# Autodesk Inventor assembly: ASY PNS-Filter column D1000
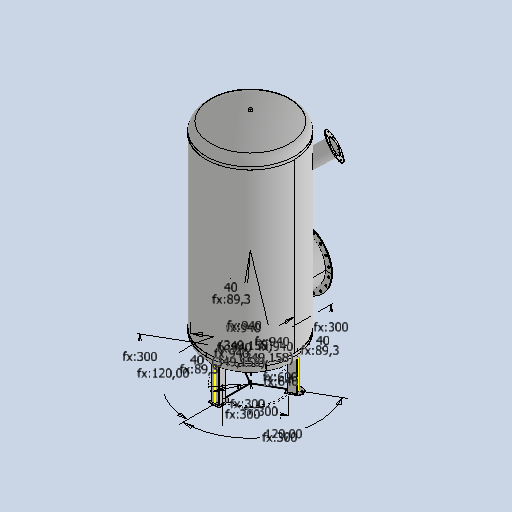
[picture p0: Inventor's stored thumbnail of the model, 512x512]
Saved by Autodesk Inventor 2025 (Build 290162010, 162A)
## iProperties
Created: 2025-02-13
Part Number: ASY PNS-Filter column D1000
Document SubType Name: Assembly
Designer: pokla
Author: pokla
Revision Number: 3
## Documents named in this file (15)
- C:\Users\admin\YandexDisk-badmisterfox\home pc\Inventor\PNS-Panaevsk\Filter D1200\ASY PNS-Filter column D1000.iam
- C:\Users\admin\YandexDisk-badmisterfox\home pc\Inventor\PNS-Panaevsk\D1000\PNS-621 charging hatch D1000.ipt
- C:\Users\admin\YandexDisk-badmisterfox\home pc\Inventor\PNS-Panaevsk\D1000\PNS-612 accses hatch flangeipt.ipt
- C:\Users\admin\YandexDisk-badmisterfox\home pc\Inventor\PNS-Panaevsk\D1000\000 DIM PNS600-Filter column D1000.ipt
- C:\Users\admin\YandexDisk-badmisterfox\home pc\Inventor\PNS-Panaevsk\D1000\PNS-611 accses hatch tube.ipt
- C:\Users\admin\YandexDisk-badmisterfox\home pc\Inventor\PNS-Panaevsk\D1000\PNS-601 main tube D1000.ipt
- C:\Users\admin\YandexDisk-badmisterfox\home pc\Inventor\PNS-Panaevsk\D1000\PNS- 652 tube.ipt
- C:\Users\admin\YandexDisk-badmisterfox\home pc\Inventor\PNS-Panaevsk\D1000\PNS-633 charging blind flange.ipt
- C:\Users\admin\YandexDisk-badmisterfox\home pc\Inventor\PNS-Panaevsk\D1000\PNS - 604 dished head D1000.ipt
- C:\Users\admin\YandexDisk-badmisterfox\home pc\Inventor\PNS-Panaevsk\Filter D1200\Fitting G1.ipt
- C:\Users\admin\YandexDisk-badmisterfox\home pc\Inventor\PNS-Panaevsk\D1000\PNS- 623 charging half tube.ipt
- C:\Users\admin\YandexDisk-badmisterfox\home pc\Inventor\PNS-Panaevsk\CC\en-US\DIN 2576 PN 10(2)\DIN 2576 Slip-On Flange for Welding Series 1 (ISO) - PN 10 500 x 508.ipt
- C:\Users\admin\YandexDisk-badmisterfox\home pc\Inventor\PNS-Panaevsk\D1000\ASY PNS680-Filter legs D1000.iam
- C:\Users\admin\YandexDisk-badmisterfox\home pc\Inventor\PNS-Panaevsk\CC\en-US\DIN 2576 PN 10(2)\DIN 2576 Slip-On Flange for Welding Series 1 (ISO) - PN 10 80 x 88.9.ipt
- C:\Users\admin\YandexDisk-badmisterfox\home pc\Inventor\PNS-Panaevsk\Filter D1200\PNS-733 charging flange round.ipt
## Components (22 placed, 14 different names)
1. 000 DIM PNS600-Filter column D1200.ipt:1
2. PNS-621 charging hatch D1200.ipt:1 — Rigid:29
3. PNS-612 accses hatch flangeipt.ipt:1 — Rigid:24, Rigid:25, Rigid:27, Rigid:28
4. PNS-611 accses hatch tube.ipt:1 — Rigid:10, Rigid:27
5. PNS-601 main tube D1000.ipt:1 — Rigid:10, Rigid:13, Rigid:14, Mate:1, Mate:2, Rigid:31, Rigid:32, Rigid:33
6. PNS- 652 tube.ipt:1 — Rotational:2, Rigid:32
7. PNS-612 accses hatch flangeipt.ipt:2 — Rigid:24, Rigid:26
8. PNS-633 charging blind flange.ipt:1
9. PNS- 652 tube.ipt:2 — Rotational:1, Rigid:33
10. PNS - 604 dished head D1200.ipt:1 — Rigid:13, Rigid:16
11. PNS - 604 dished head D1200.ipt:2 — Rigid:14, Rigid:15, Mate:3
12. Fitting G1.ipt:1 — Rigid:15
13. Fitting G1.ipt:2 — Rigid:16
14. PNS- 623 charging half tube.ipt:2 — Rigid:31, Rigid:34
15. PNS-633 charging blind flange.ipt:2
16. DIN 2576 Slip-On Flange for Welding Series 1 (ISO) - PN 10 500 x 508.ipt:1 — Rigid:28
17. PNS-612 accses hatch flangeipt.ipt:3 — Rigid:25, Rigid:29
18. PNS-612 accses hatch flangeipt.ipt:4 — Rigid:26
19. ASY PNS680-Filter legs D1200.iam:1 [sub-assembly] — Mate:4, Flush:2, Mate:5
20. DIN 2576 Slip-On Flange for Welding Series 1 (ISO) - PN 10 80 x 88.9.ipt:1 — Rotational:2
21. DIN 2576 Slip-On Flange for Welding Series 1 (ISO) - PN 10 80 x 88.9.ipt:2 — Rotational:1
22. PNS-733 charging flange round:1 — Rigid:34
## Relationships (23: WeldJoint 15, Mate 5, RevoluteJoint 2, Flush 1)
- Rigid:10 [WeldJoint] (66 mm): PNS-611 accses hatch tube.ipt:1 ↔ PNS-601 main tube D1000.ipt:1
- Rigid:13 [WeldJoint]: PNS-601 main tube D1000.ipt:1 ↔ PNS - 604 dished head D1200.ipt:1
- Rigid:14 [WeldJoint]: PNS-601 main tube D1000.ipt:1 ↔ PNS - 604 dished head D1200.ipt:2
- Rigid:15 [WeldJoint]: PNS - 604 dished head D1200.ipt:2 ↔ Fitting G1.ipt:1
- Rigid:16 [WeldJoint]: PNS - 604 dished head D1200.ipt:1 ↔ Fitting G1.ipt:2
- Rigid:24 [WeldJoint]: PNS-612 accses hatch flangeipt.ipt:1 ↔ PNS-612 accses hatch flangeipt.ipt:2
- Rigid:25 [WeldJoint]: PNS-612 accses hatch flangeipt.ipt:1 ↔ PNS-612 accses hatch flangeipt.ipt:3
- Rigid:26 [WeldJoint]: PNS-612 accses hatch flangeipt.ipt:2 ↔ PNS-612 accses hatch flangeipt.ipt:4
- Rigid:27 [WeldJoint]: PNS-612 accses hatch flangeipt.ipt:1 ↔ PNS-611 accses hatch tube.ipt:1
- Rigid:28 [WeldJoint]: PNS-612 accses hatch flangeipt.ipt:1 ↔ DIN 2576 Slip-On Flange for Welding Series 1 (ISO) - PN 10 500 x 508.ipt:1
- Mate:1: PNS-601 main tube D1000.ipt:1
- Mate:2: PNS-601 main tube D1000.ipt:1
- Mate:3 (2540 mm): PNS - 604 dished head D1200.ipt:2
- Mate:4: ASY PNS680-Filter legs D1200.iam:1
- Flush:2: ASY PNS680-Filter legs D1200.iam:1
- Mate:5: ASY PNS680-Filter legs D1200.iam:1
- Rigid:29 [WeldJoint]: PNS-621 charging hatch D1200.ipt:1 ↔ PNS-612 accses hatch flangeipt.ipt:3
- Rotational:1 [RevoluteJoint]: PNS- 652 tube.ipt:2 ↔ DIN 2576 Slip-On Flange for Welding Series 1 (ISO) - PN 10 80 x 88.9.ipt:2
- Rotational:2 [RevoluteJoint]: PNS- 652 tube.ipt:1 ↔ DIN 2576 Slip-On Flange for Welding Series 1 (ISO) - PN 10 80 x 88.9.ipt:1
- Rigid:31 [WeldJoint]: PNS-601 main tube D1000.ipt:1 ↔ PNS- 623 charging half tube.ipt:2
- Rigid:32 [WeldJoint]: PNS-601 main tube D1000.ipt:1 ↔ PNS- 652 tube.ipt:1
- Rigid:33 [WeldJoint]: PNS-601 main tube D1000.ipt:1 ↔ PNS- 652 tube.ipt:2
- Rigid:34 [WeldJoint]: PNS- 623 charging half tube.ipt:2 ↔ PNS-733 charging flange round:1
